# Autodesk Inventor assembly: Assembly_Lens_XY_Translator
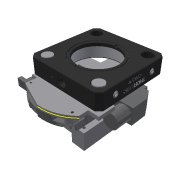
[picture p0: Inventor's stored thumbnail of the model, 180x180]
Saved by Autodesk Inventor 2019 (Build 230136000, 136)
## iProperties
Created: 2018-10-06
Part Number: Assembly_Lens_XY_Translator
Document SubType Name: Assembly
Designer: diederichbenedict
Author: diederichbenedict
## Documents named in this file (4)
- C:\Users\diederichbenedict\Dropbox\Dokumente\Promotion\PROJECTS\STORMoChip\INVENTOR\Workspaces\Arbeitsbereich\10_Cube_Base\Assembly_Lens_XY_Translator.iam
- C:\Users\diederichbenedict\Dropbox\Dokumente\Promotion\PROJECTS\STORMoChip\INVENTOR\Workspaces\Arbeitsbereich\10_Cube_Base\CP02_M-Step.ipt
- C:\Users\diederichbenedict\Dropbox\Dokumente\Promotion\PROJECTS\STORMoChip\INVENTOR\Workspaces\Arbeitsbereich\10_Cube_Base\Assembly_China_XY_Table.iam
- C:\Users\diederichbenedict\Dropbox\Dokumente\Promotion\PROJECTS\STORMoChip\INVENTOR\Workspaces\Arbeitsbereich\10_Cube_Base\00_Adapter_Lens_PCB_XY_Translator.ipt
## Components (3 placed, 3 different names)
1. Assembly_China_XY_Table:1 [sub-assembly] — Mate:1, Mate:2, Mate:3
2. CP02_M-Step:1 — Mate:1, Mate:2, Mate:3
3. 00_Adapter_Lens_PCB_XY_Translator:1
## Relationships (4: Mate 3, Flush 1)
- Mate:1 (3 mm): Assembly_China_XY_Table:1 ↔ CP02_M-Step:1
- Mate:2: Assembly_China_XY_Table:1 ↔ CP02_M-Step:1
- Mate:3: Assembly_China_XY_Table:1 ↔ CP02_M-Step:1
- [Flush]: Assembly_China_XY_Table:1 ↔ 00_Adapter_Lens_PCB_XY_Translator:1
